# Autodesk Inventor assembly: BRACER ASSEMBLIES
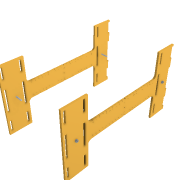
[picture p0: Inventor's stored thumbnail of the model, 180x180]
Saved by Autodesk Inventor 2022.3 (Build 263350030, 350C)
## iProperties
Created: 2021-06-17
Part Number: BRACER ASSEMBLIES
Document SubType Name: Assembly
Designer: benka
Author: benka
## Documents named in this file (3)
- C:\Users\benka\University College London\AHRC - PBD Exhibitions - UCL_Code(Development) - UCL_Code(All)\0.Board Manufacturing&Box building\1.In-home manufacturing\PBD case\UIST Case\Model\BRACER ASSEMBLIES.iam
- C:\Users\benka\University College London\AHRC - PBD Exhibitions - UCL_Code(Development) - UCL_Code(All)\0.Board Manufacturing&Box building\1.In-home manufacturing\PBD case\UIST Case\Model\ipt\side bracer.ipt
- C:\Users\benka\University College London\AHRC - PBD Exhibitions - UCL_Code(Development) - UCL_Code(All)\0.Board Manufacturing&Box building\1.In-home manufacturing\PBD case\UIST Case\Model\ipt\M4 Hex Screw v2 - 25.ipt
## Components (6 placed, 2 different names)
1. side bracer:1 — Insert:1, Insert:2
2. side bracer:2
3. M4 Hex Screw v2 - 25:3
4. M4 Hex Screw v2 - 25:4
5. M4 Hex Screw v2 - 25:5 — Insert:1
6. M4 Hex Screw v2 - 25:6 — Insert:2
## Relationships (2: Insert 2)
- Insert:1: side bracer:1 ↔ M4 Hex Screw v2 - 25:5
- Insert:2: side bracer:1 ↔ M4 Hex Screw v2 - 25:6
